# Autodesk Inventor assembly: Carril
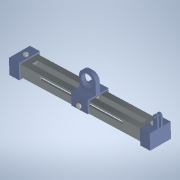
[picture p0: Inventor's stored thumbnail of the model, 180x180]
Saved by Autodesk Inventor 2022 (Build 260153000, 153)
## iProperties
Created: 2022-01-30
Part Number: Carril
Document SubType Name: Assembly
Designer: katha
Author: katha
## Documents named in this file (8)
- C:\Users\katha\OneDrive\Escritorio\Mini_Proyecto_Diseno\Diseno_18012\Modelo_MPD\Carril.iam
- C:\Users\katha\OneDrive\Escritorio\Mini_Proyecto_Diseno\Diseno_18012\Modelo_MPD\Lateral_Carril.ipt
- C:\Users\katha\OneDrive\Escritorio\Mini_Proyecto_Diseno\Diseno_18012\Modelo_MPD\Base_Carril.ipt
- C:\Users\katha\OneDrive\Escritorio\Mini_Proyecto_Diseno\Diseno_18012\Modelo_MPD\Tope_Carril.ipt
- C:\Users\katha\OneDrive\Escritorio\Mini_Proyecto_Diseno\Diseno_18012\Modelo_MPD\Tope_Carril_derecho.ipt
- C:\Users\katha\OneDrive\Escritorio\Mini_Proyecto_Diseno\Diseno_18012\Modelo_MPD\Eje_Carril.ipt
- C:\Users\katha\OneDrive\Escritorio\Mini_Proyecto_Diseno\Diseno_18012\Modelo_MPD\M4_short.ipt
- C:\Users\katha\OneDrive\Escritorio\Mini_Proyecto_Diseno\Diseno_18012\Modelo_MPD\M4_tuerca.ipt
## Components (14 placed, 7 different names)
1. Lateral_Carril:1 — Flush:1, Flush:3, Mate:2, Mate:4, Mate:7, Mate:18, Mate:19, Mate:30
2. Lateral_Carril:2 — Flush:2, Flush:4, Mate:1, Mate:10, Mate:28
3. Base_Carril:1 — Flush:1, Flush:2, Flush:3, Flush:4, Mate:1, Mate:2, Mate:3, Mate:5, Mate:6, Mate:8, Mate:17
4. Tope_Carril:1 — Mate:3, Mate:4, Mate:5, Mate:21, Mate:24, Mate:34
5. Tope_Carril_derecho:1 — Mate:6, Mate:7, Mate:8, Mate:22, Mate:23, Mate:32
6. Eje_Carril:1 — Mate:10, Mate:17, Mate:18, Mate:20, Mate:25, Mate:26
7. M4_short:1 — Mate:20, Mate:26, Mate:27
8. M4_short:2 — Mate:19, Mate:25, Mate:29
9. M4_short:3 — Mate:22, Mate:23, Mate:31
10. M4_short:4 — Mate:21, Mate:24, Mate:33
11. M4_tuerca:1 — Mate:33, Mate:34
12. M4_tuerca:2 — Mate:31, Mate:32
13. M4_tuerca:3 — Mate:29, Mate:30
14. M4_tuerca:4 — Mate:27, Mate:28
## Relationships (31: Mate 27, Flush 4)
- Flush:1: Lateral_Carril:1 ↔ Base_Carril:1
- Flush:2: Lateral_Carril:2 ↔ Base_Carril:1
- Flush:3: Lateral_Carril:1 ↔ Base_Carril:1
- Flush:4: Lateral_Carril:2 ↔ Base_Carril:1
- Mate:1: Lateral_Carril:2 ↔ Base_Carril:1
- Mate:2: Lateral_Carril:1 ↔ Base_Carril:1
- Mate:3 (0.3 mm): Base_Carril:1 ↔ Tope_Carril:1
- Mate:4: Lateral_Carril:1 ↔ Tope_Carril:1
- Mate:5: Base_Carril:1 ↔ Tope_Carril:1
- Mate:6 (0.3 mm): Base_Carril:1 ↔ Tope_Carril_derecho:1
- Mate:7: Lateral_Carril:1 ↔ Tope_Carril_derecho:1
- Mate:8: Base_Carril:1 ↔ Tope_Carril_derecho:1
- Mate:10 (0.3 mm): Lateral_Carril:2 ↔ Eje_Carril:1
- Mate:17 (0.2 mm): Base_Carril:1 ↔ Eje_Carril:1
- Mate:18 (0.119 mm): Lateral_Carril:1 ↔ Eje_Carril:1
- Mate:19: Lateral_Carril:1 ↔ M4_short:2
- Mate:20: Eje_Carril:1 ↔ M4_short:1
- Mate:21: Tope_Carril:1 ↔ M4_short:4
- Mate:22: Tope_Carril_derecho:1 ↔ M4_short:3
- Mate:23: Tope_Carril_derecho:1 ↔ M4_short:3
- Mate:24: Tope_Carril:1 ↔ M4_short:4
- Mate:25: Eje_Carril:1 ↔ M4_short:2
- Mate:26: Eje_Carril:1 ↔ M4_short:1
- Mate:27: M4_short:1 ↔ M4_tuerca:4
- Mate:28: Lateral_Carril:2 ↔ M4_tuerca:4
- Mate:29: M4_short:2 ↔ M4_tuerca:3
- Mate:30: Lateral_Carril:1 ↔ M4_tuerca:3
- Mate:31: M4_short:3 ↔ M4_tuerca:2
- Mate:32: Tope_Carril_derecho:1 ↔ M4_tuerca:2
- Mate:33: M4_short:4 ↔ M4_tuerca:1
- Mate:34: Tope_Carril:1 ↔ M4_tuerca:1
